# Autodesk Inventor assembly: cylinder
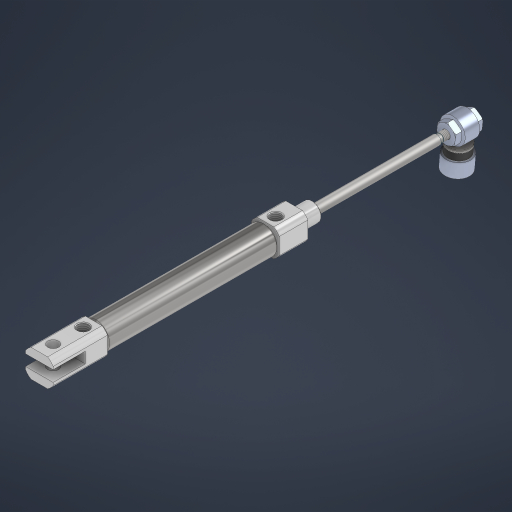
[picture p0: Inventor's stored thumbnail of the model, 512x512]
Saved by Autodesk Inventor 2024 (Build 280153000, 153)
## iProperties
Created: 2023-11-08
Part Number: cylinder
Document SubType Name: Assembly
Designer: avere
Author: avere
## Documents named in this file (9)
- C:\Users\avere\Documents\rbp_cad\zoomba_v0.1\chassis\wing\cylinder.iam
- C:\Users\avere\Documents\rbp_cad\VEX-CAD-Inventor-1.41\Motion\Pneumatics\Double Acting Piston.iam
- C:\Users\avere\Documents\rbp_cad\VEX-CAD-Inventor-1.41\Motion\Shaft LS\Shaft Collar ipts\Shaft Collar No Screw.ipt
- C:\Users\avere\Documents\rbp_cad\VEX-CAD-Inventor-1.41\Motion\Pneumatics\Piston Nut.ipt
- C:\Users\avere\Documents\rbp_cad\VEX-CAD-Inventor-1.41\Motion\Spacers\Washer Steel\SWasher .375 OD x .031250.ipt
- C:\Users\avere\Documents\rbp_cad\VEX-CAD-Inventor-1.41\Motion\Spacers\Washer Steel.ipt
- C:\Users\avere\Documents\rbp_cad\VEX-CAD-Inventor-1.41\Motion\Spacers\Washer Steel\SWasher .375 OD x .015625.ipt
- C:\Users\avere\Documents\rbp_cad\VEX-CAD-Inventor-1.41\Motion\Spacers\Spacer Nylon .375 OD\NSpacer .375 OD x .125.ipt
- C:\Users\avere\Documents\rbp_cad\VEX-CAD-Inventor-1.41\Motion\Spacers\Spacer Nylon .375 OD.ipt
## Components (8 placed, 6 different names)
1. Double Acting Piston:1 [sub-assembly] — Angle:1
2. Shaft Collar No Screw:1
3. Shaft Collar No Screw:2
4. Piston Nut:1
5. Piston Nut:2
6. SWasher .375 OD x .031250:2
7. SWasher .375 OD x .015625:3
8. NSpacer .375 OD x .125:1
## Relationships (9: Insert 6, Mate 2, Angle 1)
- [Mate]: Double Acting Piston:1 ↔ Shaft Collar No Screw:1
- [Insert] (3.175 mm): Double Acting Piston:1 ↔ Shaft Collar No Screw:1
- [Mate]: Shaft Collar No Screw:1 ↔ Shaft Collar No Screw:2
- [Insert]: Shaft Collar No Screw:1 ↔ Piston Nut:1
- [Insert]: Shaft Collar No Screw:1 ↔ Piston Nut:2
- [Insert]: SWasher .375 OD x .031250:2 ↔ SWasher .375 OD x .015625:3
- [Insert]: SWasher .375 OD x .031250:2 ↔ NSpacer .375 OD x .125:1
- [Insert]: Shaft Collar No Screw:2 ↔ NSpacer .375 OD x .125:1
- Angle:1 (0 deg): Double Acting Piston:1
